# Autodesk Inventor assembly: Drive
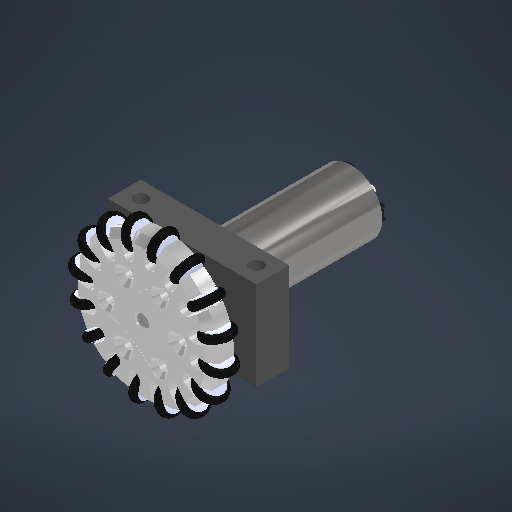
[picture p0: Inventor's stored thumbnail of the model, 512x512]
Saved by Autodesk Inventor 2025.2 (Build 292293000, 293)
## iProperties
Created: 2023-05-12
Part Number: Drive
Document SubType Name: Assembly
Designer: Elias Braun
Author: Elias Braun
## Documents named in this file (4)
- C:\Users\EliasBraun\Nextcloud2\RoboCup2023 - WM\Motor\Drive.iam
- C:\Users\EliasBraun\Nextcloud2\RoboCup2023 - WM\Motor\MotorBracket.ipt
- C:\Users\EliasBraun\Nextcloud2\RoboCup2023 - WM\Motor\Maxon\B7B9384D898D.iam
- C:\Users\EliasBraun\Nextcloud2\RoboCup2023 - WM\Motor\Wheel\Rad.iam
## Components (3 placed, 3 different names)
1. MotorBracket:1 — Mate:1, Mate:2, Mate:3, Mate:5
2. B7B9384D898D:1 [sub-assembly] — Mate:1, Mate:2, Mate:3, Mate:4
3. Rad:1 [sub-assembly] — Mate:4, Mate:5
## Relationships (5: Mate 5)
- Mate:1: MotorBracket:1 ↔ B7B9384D898D:1
- Mate:2: MotorBracket:1 ↔ B7B9384D898D:1
- Mate:3: MotorBracket:1 ↔ B7B9384D898D:1
- Mate:4: B7B9384D898D:1 ↔ Rad:1
- Mate:5: MotorBracket:1 ↔ Rad:1
